# Autodesk Inventor assembly: base Plate Laser Full Carou ASSEMBLY
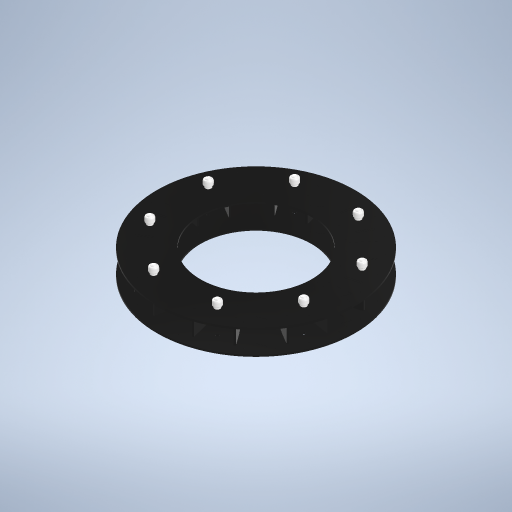
[picture p0: Inventor's stored thumbnail of the model, 512x512]
Saved by Autodesk Inventor 2023 (Build 270158000, 158)
## iProperties
Created: 2023-02-13
Part Number: base Plate Laser Full Carou ASSEMBLY
Document SubType Name: Assembly
Designer: cheng
Author: cheng
## Documents named in this file (2)
- C:\Users\cheng\Desktop\4th Year Project\Inventor\12th Assembly\Carousel Base Plate Laser Cut\base Plate Laser Full Carou ASSEMBLY.iam
- C:\Users\cheng\Desktop\4th Year Project\Inventor\12th Assembly\Carousel Base Plate Laser Cut\Base Plate Laser Assembly.iam
## Components (8 placed, 1 different names)
1. Base Plate Laser Assembly:1 [sub-assembly] — Mate:7, Flush:4, Mate:8
2. Base Plate Laser Assembly:2 [sub-assembly] — Mate:13, Mate:14, Flush:7
3. Base Plate Laser Assembly:3 [sub-assembly] — Mate:9, Mate:10, Flush:5, Mate:11, Mate:12, Flush:6
4. Base Plate Laser Assembly:4 [sub-assembly] — Mate:11, Mate:12, Flush:6, Mate:13, Mate:14, Flush:7
5. Base Plate Laser Assembly:5 [sub-assembly] — Flush:2, Mate:3, Mate:4, Mate:5, Flush:3, Mate:6
6. Base Plate Laser Assembly:6 [sub-assembly] — Mate:5, Flush:3, Mate:6, Mate:7, Flush:4, Mate:8
7. Base Plate Laser Assembly:7 [sub-assembly] — Mate:1, Mate:2, Flush:1, Mate:9, Mate:10, Flush:5
8. Base Plate Laser Assembly:8 [sub-assembly] — Mate:1, Mate:2, Flush:1, Flush:2, Mate:3, Mate:4
## Relationships (21: Mate 14, Flush 7)
- Mate:1: Base Plate Laser Assembly:7 ↔ Base Plate Laser Assembly:8
- Mate:2: Base Plate Laser Assembly:7 ↔ Base Plate Laser Assembly:8
- Flush:1: Base Plate Laser Assembly:7 ↔ Base Plate Laser Assembly:8
- Flush:2: Base Plate Laser Assembly:5 ↔ Base Plate Laser Assembly:8
- Mate:3: Base Plate Laser Assembly:5 ↔ Base Plate Laser Assembly:8
- Mate:4: Base Plate Laser Assembly:5 ↔ Base Plate Laser Assembly:8
- Mate:5: Base Plate Laser Assembly:5 ↔ Base Plate Laser Assembly:6
- Flush:3: Base Plate Laser Assembly:5 ↔ Base Plate Laser Assembly:6
- Mate:6: Base Plate Laser Assembly:5 ↔ Base Plate Laser Assembly:6
- Mate:7: Base Plate Laser Assembly:1 ↔ Base Plate Laser Assembly:6
- Flush:4: Base Plate Laser Assembly:1 ↔ Base Plate Laser Assembly:6
- Mate:8: Base Plate Laser Assembly:1 ↔ Base Plate Laser Assembly:6
- Mate:9: Base Plate Laser Assembly:3 ↔ Base Plate Laser Assembly:7
- Mate:10: Base Plate Laser Assembly:3 ↔ Base Plate Laser Assembly:7
- Flush:5: Base Plate Laser Assembly:3 ↔ Base Plate Laser Assembly:7
- Mate:11: Base Plate Laser Assembly:3 ↔ Base Plate Laser Assembly:4
- Mate:12: Base Plate Laser Assembly:3 ↔ Base Plate Laser Assembly:4
- Flush:6: Base Plate Laser Assembly:3 ↔ Base Plate Laser Assembly:4
- Mate:13: Base Plate Laser Assembly:2 ↔ Base Plate Laser Assembly:4
- Mate:14: Base Plate Laser Assembly:2 ↔ Base Plate Laser Assembly:4
- Flush:7: Base Plate Laser Assembly:2 ↔ Base Plate Laser Assembly:4
